# Autodesk Inventor assembly: Bumpers
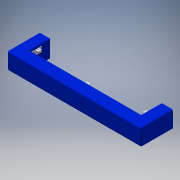
[picture p0: Inventor's stored thumbnail of the model, 180x180]
Saved by Autodesk Inventor 2016 (Build 200138000, 138)
## iProperties
Created: 2017-01-28
Part Number: Bumpers
Document SubType Name: Assembly
Designer: hamblettk
Author: hamblettk
## Documents named in this file (3)
- E:\1073CAD\Robot2017\DriveTrain\Let's try this again\Bumpers.iam
- E:\1073CAD\Robot2017\DriveTrain\Let's try this again\Bumper.ipt
- E:\1073CAD\Robot2017\DriveTrain\Let's try this again\BumperBracket.ipt
## Components (4 placed, 2 different names)
1. Bumper:1 — Mate:1, Mate:2, Mate:3, Flush:1, Mate:4, Flush:6, Flush:7, Flush:8, Flush:9
2. BumperBracket:1 — Mate:3, Flush:6, Flush:9
3. BumperBracket:2 — Mate:2, Mate:4, Flush:8
4. BumperBracket:3 — Mate:1, Flush:1, Flush:7
## Relationships (9: Flush 5, Mate 4)
- Mate:1: Bumper:1 ↔ BumperBracket:3
- Mate:2: Bumper:1 ↔ BumperBracket:2
- Mate:3: Bumper:1 ↔ BumperBracket:1
- Flush:1 (63.5 mm): Bumper:1 ↔ BumperBracket:3
- Mate:4 (374.65 mm): Bumper:1 ↔ BumperBracket:2
- Flush:6 (63.5 mm): Bumper:1 ↔ BumperBracket:1
- Flush:7 (12.7 mm): Bumper:1 ↔ BumperBracket:3
- Flush:8 (12.7 mm): Bumper:1 ↔ BumperBracket:2
- Flush:9 (12.7 mm): Bumper:1 ↔ BumperBracket:1
